# Autodesk Inventor assembly: replacementHandleStu
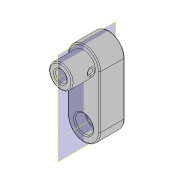
[picture p0: Inventor's stored thumbnail of the model, 180x180]
Saved by Autodesk Inventor 2021 (Build 250183000, 183)
## iProperties
Created: 2020-09-27
Part Number: replacementHandleStu
Document SubType Name: Assembly
Designer: Stu
Author: Stu
## Documents named in this file (2)
- C:\Users\Stu\Google Drive\Projects\CAD\Workmate Handle\replacementHandleStu.iam
- C:\Users\Stu\Google Drive\Projects\CAD\Workmate Handle\replacementHandleStu.ipt
## Components (1 placed, 1 different names)
1. replacementHandleStu:1 — Flush:1, Flush:2, Flush:3
## Relationships (3: Flush 3)
- Flush:1: replacementHandleStu:1
- Flush:2: replacementHandleStu:1
- Flush:3: replacementHandleStu:1
